# Autodesk Inventor assembly: Odometry module for metal drive train
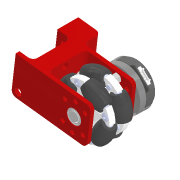
[picture p0: Inventor's stored thumbnail of the model, 180x180]
Saved by Autodesk Inventor 2020 (Build 240168000, 168)
## iProperties
Created: 2019-11-05
Part Number: Odometry module for metal drive train
Document SubType Name: Assembly
Designer: ball
Author: ball
## Documents named in this file (8)
- C:\FTC\FTC8863CAD\2019 Robot\Odoemetry module\Odometry module for metal drive train.iam
- C:\FTC\FTC8863CAD\Actobotics\535 parts\535042.ipt
- C:\FTC\FTC8863CAD\Actobotics\634 parts\634064.ipt
- C:\FTC\FTC8863CAD\2019 Robot\Odoemetry module\wheel_dual.iam
- C:\FTC\FTC8863CAD\2019 Robot\Odoemetry module\E8T-X-250-S-D-D-X.iam
- C:\FTC\FTC8863CAD\2019 Robot\Odoemetry module\90576A161_MEDIUM-STRENGTH STEEL NYLON-INSERT LOCKNUT.ipt
- C:\FTC\FTC8863CAD\2019 Robot\Odoemetry module\spacer around nuts.ipt
- C:\FTC\FTC8863CAD\2019 Robot\Odoemetry module\Odometry_Holder with motor clearance.ipt
## Components (9 placed, 7 different names)
1. Odometry_Holder with motor clearance:1 — Mate:1, Mate:2, Mate:3, Flush:1, Mate:11, Mate:12, Mate:14, Mate:16
2. 535042:1 — Mate:1, Mate:2
3. 535042:2 — Mate:3, Mate:5
4. 634064:1 — Mate:5, Flush:1, Mate:6, Mate:10, Mate:18
5. wheel_dual:1 [sub-assembly] — Mate:6, Mate:17
6. E8T-X-250-S-D-D-X:1 [sub-assembly] — Mate:10, Mate:11, Mate:12, Mate:13, Mate:15
7. 90576A161_MEDIUM-STRENGTH STEEL NYLON-INSERT LOCKNUT:1 — Mate:13, Mate:14
8. 90576A161_MEDIUM-STRENGTH STEEL NYLON-INSERT LOCKNUT:2 — Mate:15, Mate:16
9. spacer around nuts:1 — Mate:17, Mate:18
## Relationships (15: Mate 14, Flush 1)
- Mate:1: Odometry_Holder with motor clearance:1 ↔ 535042:1
- Mate:2: Odometry_Holder with motor clearance:1 ↔ 535042:1
- Mate:3: Odometry_Holder with motor clearance:1 ↔ 535042:2
- Mate:5: 535042:2 ↔ 634064:1
- Flush:1: Odometry_Holder with motor clearance:1 ↔ 634064:1
- Mate:6: 634064:1 ↔ wheel_dual:1
- Mate:10: 634064:1 ↔ E8T-X-250-S-D-D-X:1
- Mate:11: Odometry_Holder with motor clearance:1 ↔ E8T-X-250-S-D-D-X:1
- Mate:12: Odometry_Holder with motor clearance:1 ↔ E8T-X-250-S-D-D-X:1
- Mate:13: E8T-X-250-S-D-D-X:1 ↔ 90576A161_MEDIUM-STRENGTH STEEL NYLON-INSERT LOCKNUT:1
- Mate:14: Odometry_Holder with motor clearance:1 ↔ 90576A161_MEDIUM-STRENGTH STEEL NYLON-INSERT LOCKNUT:1
- Mate:15: E8T-X-250-S-D-D-X:1 ↔ 90576A161_MEDIUM-STRENGTH STEEL NYLON-INSERT LOCKNUT:2
- Mate:16: Odometry_Holder with motor clearance:1 ↔ 90576A161_MEDIUM-STRENGTH STEEL NYLON-INSERT LOCKNUT:2
- Mate:17: wheel_dual:1 ↔ spacer around nuts:1
- Mate:18: 634064:1 ↔ spacer around nuts:1
